# Autodesk Inventor assembly: MX-28T_R+idle.ipt
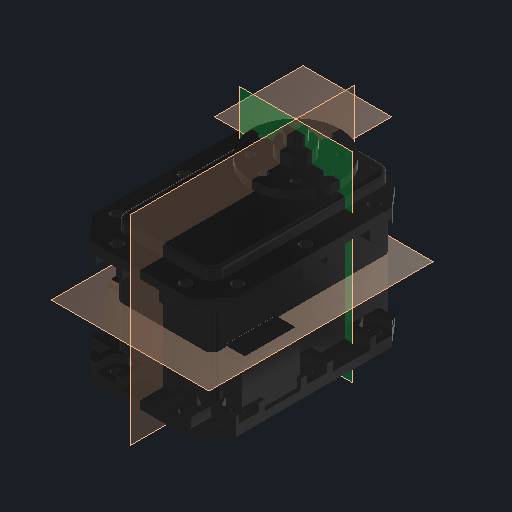
[picture p0: Inventor's stored thumbnail of the model, 512x512]
Saved by Autodesk Inventor 2024 (Build 280153000, 153)
## iProperties
Created: 2022-08-09
Part Number: MX-28T_R+idle.ipt
Document SubType Name: Assembly
Designer: 박지훈
Mass: 83 g
Surface Area: 131.328 cm^2
Volume: 44.8383 cm^3
Density: 1.8511 g/cm^3
Author: 박지훈
## Documents named in this file (3)
- C:\Users\USER\Desktop\2024_Robit_Hardware\ROBOCUP_2024_eindhoven\부품\ROBOTIS(Inventor 2023 ver.)\다이나믹셀\MX-28T_R+idle.ipt.iam
- C:\Users\USER\Desktop\2024_Robit_Hardware\ROBOCUP_2024_eindhoven\부품\ROBOTIS(Inventor 2023 ver.)\아이들러\28아이들러.iam
- C:\Users\USER\Desktop\2024_Robit_Hardware\ROBOCUP_2024_eindhoven\부품\ROBOTIS(Inventor 2023 ver.)\다이나믹셀\MX-28T_R.ipt
## Components (2 placed, 2 different names)
1. 28아이들러:1 [sub-assembly] — 삽입:1
2. MX-28T_R:1 — 삽입:1
## Relationships (1: Insert 1)
- 삽입:1 [Insert] (0.1 mm): 28아이들러:1 ↔ MX-28T_R:1
